# Autodesk Inventor assembly: ギアボックス
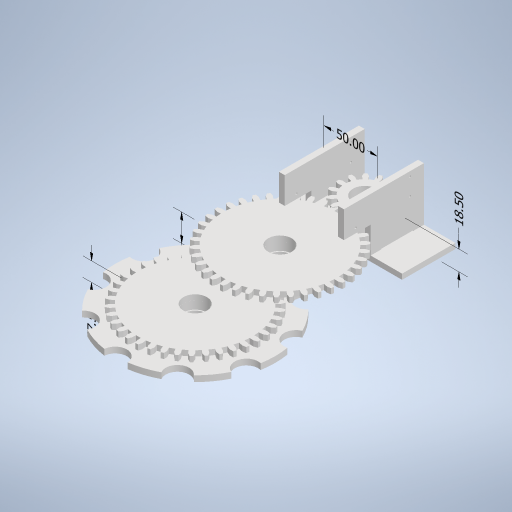
[picture p0: Inventor's stored thumbnail of the model, 512x512]
Saved by Autodesk Inventor 2024.1 (Build 281209000, 209)
## iProperties
Created: 2024-04-01
Part Number: ギアボックス
Document SubType Name: Assembly
Designer: hibik
Author: hibik
## Documents named in this file (9)
- C:\Users\hibik\Desktop\ロボメカ\2年\新歓\ベルトコンベア\ギアボックス.iam
- C:\Users\hibik\Desktop\ロボメカ\2年\新歓\ベルトコンベア\ギアプレート.ipt
- C:\Users\hibik\Desktop\ロボメカ\2年\新歓\ベルトコンベア\M15_10.ipt
- C:\Users\hibik\Desktop\ロボメカ\2年\新歓\ベルトコンベア\M3_38.ipt
- C:\Users\hibik\Desktop\ロボメカ\2年\新歓\ベルトコンベア\M3_15.ipt
- C:\Users\hibik\Desktop\ロボメカ\2年\新歓\ベルトコンベア\spacer.ipt
- C:\Users\hibik\Desktop\ロボメカ\2年\新歓\ベルトコンベア\ギアプレートupper.ipt
- C:\Users\hibik\Desktop\ロボメカ\2年\新歓\ベルトコンベア\ギアプレートupper_upper.ipt
- C:\Users\hibik\Desktop\ロボメカ\2年\新歓\ベルトコンベア\壁.ipt
## Components (13 placed, 8 different names)
1. ギアプレート:1 — 挿入:4, 挿入:6, 挿入:7, フラッシュ:3, フラッシュ:4, フラッシュ:5, フラッシュ:6, メイト:1, メイト:2
2. M15_10:1 — 挿入:2, 挿入:5
3. M3_38:1 — 挿入:2
4. M3_38:2 — 挿入:3
5. M3_15:1 — 挿入:3, 挿入:9
6. M3_15:2 — 挿入:13
7. spacer:1 — 挿入:4, 挿入:5
8. spacer:2 — 挿入:8, 挿入:9, 挿入:10
9. ギアプレートupper:1 — 挿入:6, 挿入:7, 挿入:8, 挿入:11
10. ギアプレートupper_upper:1 — 挿入:10, 挿入:11, 挿入:12
11. spacer:3 — 挿入:12, 挿入:13
12. 壁:1 — フラッシュ:4, フラッシュ:6, メイト:1
13. 壁:2 — フラッシュ:3, フラッシュ:5, メイト:2
## Relationships (18: Insert 12, Flush 4, Mate 2)
- 挿入:2 [Insert]: M15_10:1 ↔ M3_38:1
- 挿入:3 [Insert]: M3_38:2 ↔ M3_15:1
- 挿入:4 [Insert]: ギアプレート:1 ↔ spacer:1
- 挿入:5 [Insert]: M15_10:1 ↔ spacer:1
- 挿入:6 [Insert]: ギアプレート:1 ↔ ギアプレートupper:1
- 挿入:7 [Insert]: ギアプレート:1 ↔ ギアプレートupper:1
- 挿入:8 [Insert]: spacer:2 ↔ ギアプレートupper:1
- 挿入:9 [Insert]: M3_15:1 ↔ spacer:2
- 挿入:10 [Insert]: spacer:2 ↔ ギアプレートupper_upper:1
- 挿入:11 [Insert]: ギアプレートupper:1 ↔ ギアプレートupper_upper:1
- 挿入:12 [Insert]: ギアプレートupper_upper:1 ↔ spacer:3
- 挿入:13 [Insert]: M3_15:2 ↔ spacer:3
- フラッシュ:3 [Flush]: ギアプレート:1 ↔ 壁:2
- フラッシュ:4 [Flush]: ギアプレート:1 ↔ 壁:1
- フラッシュ:5 [Flush]: ギアプレート:1 ↔ 壁:2
- フラッシュ:6 [Flush]: ギアプレート:1 ↔ 壁:1
- メイト:1 [Mate]: ギアプレート:1 ↔ 壁:1
- メイト:2 [Mate]: ギアプレート:1 ↔ 壁:2
